# Autodesk Inventor assembly: Drive
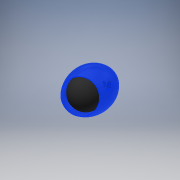
[picture p0: Inventor's stored thumbnail of the model, 180x180]
Saved by Autodesk Inventor 2018.3 (Build 223284000, 284)
## iProperties
Created: 2018-06-30
Part Number: Drive
Material: Generisch
Document SubType Name: Assembly
Designer: JochenAlt
Author: JochenAlt
## Documents named in this file (5)
- D:\Projects\FlowerPot\CAD\Drive.iam
- D:\Projects\FlowerPot\CAD\DriveChain.iam
- D:\Projects\FlowerPot\CAD\Sphere.ipt
- D:\Projects\FlowerPot\CAD\Spindle\SpindleThread.ipt
- D:\Projects\FlowerPot\CAD\Form.iam
## Components (8 placed, 4 different names)
1. Antriebsstrang:1 [sub-assembly] — Passend:1, Passend:3, Passend:5, Passend:35, Passend:36, Fluchtend:1
2. Antriebsstrang:2 [sub-assembly] — Passend:2, Passend:4, Passend:34, Passend:37, Fluchtend:2
3. Antriebsstrang:3 [sub-assembly] — Passend:1, Passend:2, Passend:3, Passend:4, Passend:26, Passend:27, Passend:34, Passend:35, Tangential:1
4. Sphere:1 — Passend:5, Tangential:1, Passend:38
5. SpindleThread:1 — Passend:26, Passend:27, Passend:39
6. SpindleThread:2 — Passend:36, Fluchtend:1
7. SpindleThread:3 — Passend:37, Fluchtend:2, Passend:40
8. Form:1 [sub-assembly] — Passend:39, Passend:40
## Relationships (17: Mate 14, Flush 2, Tangent 1)
- Passend:1 [Mate]: Antriebsstrang:1 ↔ Antriebsstrang:3
- Passend:2 [Mate]: Antriebsstrang:2 ↔ Antriebsstrang:3
- Passend:3 [Mate]: Antriebsstrang:1 ↔ Antriebsstrang:3
- Passend:4 [Mate]: Antriebsstrang:2 ↔ Antriebsstrang:3
- Passend:5 [Mate]: Antriebsstrang:1 ↔ Sphere:1
- Passend:26 [Mate]: Antriebsstrang:3 ↔ SpindleThread:1
- Passend:27 [Mate]: Antriebsstrang:3 ↔ SpindleThread:1
- Passend:34 [Mate]: Antriebsstrang:2 ↔ Antriebsstrang:3
- Passend:35 [Mate]: Antriebsstrang:1 ↔ Antriebsstrang:3
- Passend:36 [Mate]: Antriebsstrang:1 ↔ SpindleThread:2
- Passend:37 [Mate]: Antriebsstrang:2 ↔ SpindleThread:3
- Fluchtend:1 [Flush]: Antriebsstrang:1 ↔ SpindleThread:2
- Fluchtend:2 [Flush]: Antriebsstrang:2 ↔ SpindleThread:3
- Tangential:1: Antriebsstrang:3 ↔ Sphere:1
- Passend:38 [Mate]: Sphere:1
- Passend:39 [Mate]: SpindleThread:1 ↔ Form:1
- Passend:40 [Mate]: SpindleThread:3 ↔ Form:1
